# Autodesk Inventor assembly: HotPlateSolderingSMD
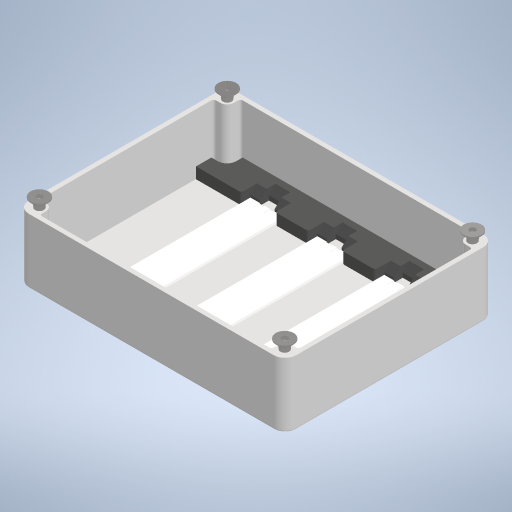
[picture p0: Inventor's stored thumbnail of the model, 512x512]
Saved by Autodesk Inventor 2024 (Build 280153000, 153)
## iProperties
Created: 2024-08-30
Part Number: HotPlateSolderingSMD
Document SubType Name: Assembly
Designer: malam
Author: malam
## Documents named in this file (6)
- C:\Users\malam\Documents\6 - PROJET\12 - HOTPLATE SOLDERING SMD\2 - CONCEPTION 3D\20 - CONCEPTION 3D\HotPlateSolderingSMD.iam
- C:\Users\malam\Documents\6 - PROJET\12 - HOTPLATE SOLDERING SMD\2 - CONCEPTION 3D\20 - CONCEPTION 3D\Boitier_aluminium.ipt
- C:\Users\malam\Documents\6 - PROJET\12 - HOTPLATE SOLDERING SMD\2 - CONCEPTION 3D\20 - CONCEPTION 3D\Couvercle_aluminium.ipt
- C:\Users\malam\Documents\6 - PROJET\12 - HOTPLATE SOLDERING SMD\2 - CONCEPTION 3D\20 - CONCEPTION 3D\Resistance_chauffante_ceramique.ipt
- C:\Users\malam\Documents\6 - PROJET\12 - HOTPLATE SOLDERING SMD\2 - CONCEPTION 3D\20 - CONCEPTION 3D\Centreur_resistance.ipt
- C:\Users\malam\Documents\6 - PROJET\12 - HOTPLATE SOLDERING SMD\2 - CONCEPTION 3D\20 - CONCEPTION 3D\BS 4168 - M4 x 16(7).ipt
## Components (11 placed, 5 different names)
1. Boitier_aluminium:1 — Placage:1, Placage:4, Placage:5, Placage:6, Placage:7, Placage:8, Placage:9, Placage:10, Placage:11, Placage:12, Placage:13, Placage:14, Placage:16, Placage:18
2. Couvercle_aluminium:1 — Placage:12, Placage:13, Placage:14, Placage:15, Affleurement:5, Placage:17, Affleurement:6, Affleurement:7, Affleurement:8
3. Resistance_chauffante_ceramique:1 — Affleurement:1, Affleurement:2, Placage:2, Affleurement:3
4. Resistance_chauffante_ceramique:2 — Affleurement:1, Placage:1, Placage:2, Placage:3, Affleurement:3, Affleurement:4, Placage:4
5. Resistance_chauffante_ceramique:3 — Affleurement:2, Placage:3, Affleurement:4, Placage:5
6. Centreur_resistance:1 — Placage:6, Placage:7, Placage:8
7. Centreur_resistance:2 — Placage:9, Placage:10, Placage:11
8. BS 4168 : Pièce 8 Vis bouton et fraisées à six pans creux - Série métrique - Métrique M4 x 16:1 — Placage:16, Affleurement:8
9. BS 4168 : Pièce 8 Vis bouton et fraisées à six pans creux - Série métrique - Métrique M4 x 16:2 — Placage:15, Affleurement:5
10. BS 4168 : Pièce 8 Vis bouton et fraisées à six pans creux - Série métrique - Métrique M4 x 16:3 — Placage:17, Affleurement:7
11. BS 4168 : Pièce 8 Vis bouton et fraisées à six pans creux - Série métrique - Métrique M4 x 16:4 — Placage:18, Affleurement:6
## Relationships (26: Mate 18, Flush 8)
- Affleurement:1 [Flush]: Resistance_chauffante_ceramique:1 ↔ Resistance_chauffante_ceramique:2
- Affleurement:2 [Flush]: Resistance_chauffante_ceramique:1 ↔ Resistance_chauffante_ceramique:3
- Placage:1 [Mate]: Boitier_aluminium:1 ↔ Resistance_chauffante_ceramique:2
- Placage:2 [Mate] (15 mm): Resistance_chauffante_ceramique:1 ↔ Resistance_chauffante_ceramique:2
- Placage:3 [Mate] (15 mm): Resistance_chauffante_ceramique:2 ↔ Resistance_chauffante_ceramique:3
- Affleurement:3 [Flush]: Resistance_chauffante_ceramique:1 ↔ Resistance_chauffante_ceramique:2
- Affleurement:4 [Flush]: Resistance_chauffante_ceramique:2 ↔ Resistance_chauffante_ceramique:3
- Placage:4 [Mate] (10 mm): Boitier_aluminium:1 ↔ Resistance_chauffante_ceramique:2
- Placage:5 [Mate] (20.5 mm): Boitier_aluminium:1 ↔ Resistance_chauffante_ceramique:3
- Placage:6 [Mate] (0.1 mm): Boitier_aluminium:1 ↔ Centreur_resistance:1
- Placage:7 [Mate] (0.1 mm): Boitier_aluminium:1 ↔ Centreur_resistance:1
- Placage:8 [Mate]: Boitier_aluminium:1 ↔ Centreur_resistance:1
- Placage:9 [Mate] (0.1 mm): Boitier_aluminium:1 ↔ Centreur_resistance:2
- Placage:10 [Mate] (0.1 mm): Boitier_aluminium:1 ↔ Centreur_resistance:2
- Placage:11 [Mate]: Boitier_aluminium:1 ↔ Centreur_resistance:2
- Placage:12 [Mate]: Boitier_aluminium:1 ↔ Couvercle_aluminium:1
- Placage:13 [Mate]: Boitier_aluminium:1 ↔ Couvercle_aluminium:1
- Placage:14 [Mate]: Boitier_aluminium:1 ↔ Couvercle_aluminium:1
- Placage:15 [Mate]: Couvercle_aluminium:1 ↔ BS 4168 : Pièce 8 Vis bouton et fraisées à six pans creux - Série métrique - Métrique M4 x 16:2
- Affleurement:5 [Flush]: Couvercle_aluminium:1 ↔ BS 4168 : Pièce 8 Vis bouton et fraisées à six pans creux - Série métrique - Métrique M4 x 16:2
- Placage:16 [Mate]: Boitier_aluminium:1 ↔ BS 4168 : Pièce 8 Vis bouton et fraisées à six pans creux - Série métrique - Métrique M4 x 16:1
- Placage:17 [Mate]: Couvercle_aluminium:1 ↔ BS 4168 : Pièce 8 Vis bouton et fraisées à six pans creux - Série métrique - Métrique M4 x 16:3
- Placage:18 [Mate]: Boitier_aluminium:1 ↔ BS 4168 : Pièce 8 Vis bouton et fraisées à six pans creux - Série métrique - Métrique M4 x 16:4
- Affleurement:6 [Flush]: Couvercle_aluminium:1 ↔ BS 4168 : Pièce 8 Vis bouton et fraisées à six pans creux - Série métrique - Métrique M4 x 16:4
- Affleurement:7 [Flush]: Couvercle_aluminium:1 ↔ BS 4168 : Pièce 8 Vis bouton et fraisées à six pans creux - Série métrique - Métrique M4 x 16:3
- Affleurement:8 [Flush]: Couvercle_aluminium:1 ↔ BS 4168 : Pièce 8 Vis bouton et fraisées à six pans creux - Série métrique - Métrique M4 x 16:1
